# Autodesk Inventor assembly: 组装
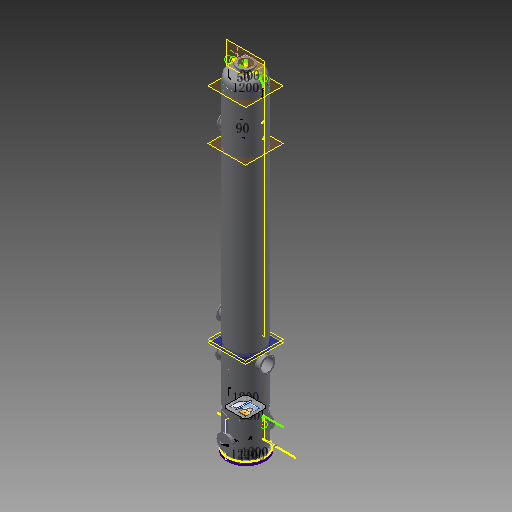
[picture p0: Inventor's stored thumbnail of the model, 512x512]
Saved by Autodesk Inventor 2018.2 (Build 222227000, 227)
## iProperties
Created: 2018-07-05
Part Number: 组装
Material: 常规
Document SubType Name: Assembly
Designer: Administrator
Author: Administrator
## Documents named in this file (11)
- C:\Users\Administrator\Desktop\填料塔\组装.iam
- C:\Users\Administrator\Desktop\填料塔\除沫器.ipt
- C:\Users\Administrator\Desktop\填料塔\结构件1.iam
- C:\Users\Administrator\Desktop\填料塔\蓬莱管.ipt
- C:\Users\Administrator\Desktop\填料塔\塔底.ipt
- C:\Users\Administrator\Desktop\填料塔\塔盖模板.ipt
- C:\Users\Administrator\Desktop\填料塔\塔体.ipt
- C:\Users\Administrator\Desktop\填料塔\支撑.ipt
- C:\Users\Administrator\Desktop\填料塔\进气孔.ipt
- C:\Users\Administrator\Desktop\填料塔\人孔.ipt
- C:\Users\Administrator\Desktop\填料塔\人孔法兰.ipt
## Components (15 placed, 10 different names)
1. 除沫器:1 — 旋转:6
2. 结构件1:1 [sub-assembly] — 旋转:3
3. 蓬莱管:1 — 刚性:2
4. 塔底:1 — 旋转:2, 旋转:3, 刚性:1, 旋转:8
5. 塔盖模板:1 — 旋转:1, 配合:1
6. 塔体:1 — 旋转:1, 旋转:2, 刚性:1, 旋转:5, 旋转:6, 旋转:7, 刚性:2, 表面齐平:1, 表面齐平:2, 刚性:8, 表面齐平:3, 刚性:9, 刚性:12, 旋转:8
7. 支撑:1 — 旋转:7
8. 支撑:2 — 旋转:5
9. 进气孔:1
10. 人孔:1 — 刚性:11, 刚性:12
11. 人孔法兰:1 — 刚性:11
12. 人孔:2 — 刚性:5, 刚性:8
13. 人孔法兰:2 — 刚性:5
14. 人孔:3 — 刚性:9
15. 人孔法兰:3
## Relationships (20: WeldJoint 8, RevoluteJoint 7, Flush 3, Mate 1, Angle 1)
- 旋转:1 [RevoluteJoint]: 塔盖模板:1 ↔ 塔体:1
- 旋转:2 [RevoluteJoint]: 塔底:1 ↔ 塔体:1
- 旋转:3 [RevoluteJoint]: 结构件1:1 ↔ 塔底:1
- 刚性:1 [WeldJoint]: 塔底:1 ↔ 塔体:1
- 配合:1 [Mate]: 塔盖模板:1
- 角度:1 [Angle] (0 deg)
- 旋转:5 [RevoluteJoint]: 塔体:1 ↔ 支撑:2
- 旋转:6 [RevoluteJoint]: 除沫器:1 ↔ 塔体:1
- 旋转:7 [RevoluteJoint]: 塔体:1 ↔ 支撑:1
- 刚性:2 [WeldJoint] (-2 mm): 蓬莱管:1 ↔ 塔体:1
- 刚性:5 [WeldJoint]: 人孔:2 ↔ 人孔法兰:2
- [WeldJoint]: 人孔:3 ↔ 人孔法兰:3
- 表面齐平:1 [Flush]: 塔体:1
- 表面齐平:2 [Flush] (-100 mm): 塔体:1
- 刚性:8 [WeldJoint] (150 mm): 塔体:1 ↔ 人孔:2
- 表面齐平:3 [Flush] (-1750 mm): 塔体:1
- 刚性:9 [WeldJoint] (150 mm): 塔体:1 ↔ 人孔:3
- 刚性:11 [WeldJoint]: 人孔:1 ↔ 人孔法兰:1
- 刚性:12 [WeldJoint] (-150 mm): 塔体:1 ↔ 人孔:1
- 旋转:8 [RevoluteJoint]: 塔底:1 ↔ 塔体:1
## Named parameters: d48_d47 = 0 mm
